# Autodesk Inventor assembly: Plate pulley v 2.0
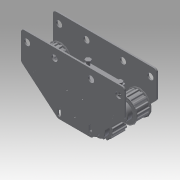
[picture p0: Inventor's stored thumbnail of the model, 180x180]
Saved by Autodesk Inventor 2016 (Build 200138000, 138)
## iProperties
Created: 2015-10-10
Part Number: Plate pulley v 2.0
Document SubType Name: Assembly
Designer: Delta
Author: Delta
## Documents named in this file (10)
- C:\Robotics\CAD\2015-16\custom cad parts\Plate pulley v 2.0.iam
- C:\Robotics\CAD\2015-16\custom cad parts\Hex standoff custom.ipt
- C:\Robotics\CAD\2015-16\custom cad parts\track side panel V1 - top hole edidtion .ipt
- C:\Robotics\CAD\2015-16\custom cad parts\wheel and axel top.iam
- C:\Robotics\CAD\2015-16\custom cad parts\wheel and axel bottom.iam
- C:\Robotics\CAD\2015-16\custom cad parts\.125 in female rod end.ipt
- C:\Robotics\CAD\2015-16\custom cad parts\1.5in bolt.ipt
- C:\Robotics\~2015-16_CAD\custom cad parts\track guide u channel middle.ipt
- C:\Robotics\~2015-16_CAD\custom cad parts\track guide u channel side.ipt
- C:\Robotics\CAD\2015-16\custom cad parts\track guide u channel.ipt
## Components (19 placed, 9 different names)
1. Hex standoff custom:2 — Insert:5
2. track side panel V1 - top hole edidtion :1 — Insert:1, Insert:2, Insert:3, Insert:4, Insert:5, Insert:16
3. wheel and axel top:1 [sub-assembly] — Insert:1, Mate:12
4. wheel and axel top:2 [sub-assembly] — Insert:2, Insert:17
5. wheel and axel bottom:1 [sub-assembly] — Insert:3, Insert:9, Insert:11
6. wheel and axel bottom:2 [sub-assembly] — Insert:4, Insert:8, Insert:10
7. .125 in female rod end:1 — Insert:9, Mate:8
8. .125 in female rod end:2 — Insert:11, Mate:6
9. .125 in female rod end:3 — Insert:8, Mate:10
10. .125 in female rod end:4 — Insert:10, Mate:5
11. 1.5in bolt:1 — Mate:6, Insert:14, Insert:18
12. 1.5in bolt:2 — Mate:10
13. 1.5in bolt:3 — Mate:8
14. 1.5in bolt:4 — Mate:5, Mate:13
15. track guide u channel middle:1 — Insert:14, Mate:11
16. track guide u channel side:1
17. track guide u channel side:2 — Mate:11, Insert:16
18. track side panel V1 - top hole edidtion :2 — Insert:17, Mate:12
19. track guide u channel:1 — Insert:18, Mate:13
## Relationships (20: Insert 13, Mate 7)
- Insert:1: track side panel V1 - top hole edidtion :1 ↔ wheel and axel top:1
- Insert:2: track side panel V1 - top hole edidtion :1 ↔ wheel and axel top:2
- Insert:3: track side panel V1 - top hole edidtion :1 ↔ wheel and axel bottom:1
- Insert:4: track side panel V1 - top hole edidtion :1 ↔ wheel and axel bottom:2
- Insert:5: Hex standoff custom:2 ↔ track side panel V1 - top hole edidtion :1
- Insert:8 (6.35 mm): wheel and axel bottom:2 ↔ .125 in female rod end:3
- Insert:9 (6.35 mm): wheel and axel bottom:1 ↔ .125 in female rod end:1
- Insert:10 (6.35 mm): wheel and axel bottom:2 ↔ .125 in female rod end:4
- Insert:11 (6.35 mm): wheel and axel bottom:1 ↔ .125 in female rod end:2
- Mate:5: .125 in female rod end:4 ↔ 1.5in bolt:4
- Mate:6: .125 in female rod end:2 ↔ 1.5in bolt:1
- Mate:8: .125 in female rod end:1 ↔ 1.5in bolt:3
- Mate:10: .125 in female rod end:3 ↔ 1.5in bolt:2
- Insert:14: 1.5in bolt:1 ↔ track guide u channel middle:1
- Mate:11: track guide u channel middle:1 ↔ track guide u channel side:2
- Insert:16: track side panel V1 - top hole edidtion :1 ↔ track guide u channel side:2
- Insert:17: wheel and axel top:2 ↔ track side panel V1 - top hole edidtion :2
- Mate:12: wheel and axel top:1 ↔ track side panel V1 - top hole edidtion :2
- Insert:18: 1.5in bolt:1 ↔ track guide u channel:1
- Mate:13: 1.5in bolt:4 ↔ track guide u channel:1
